# Autodesk Inventor assembly: Shipping goods QR subassembly
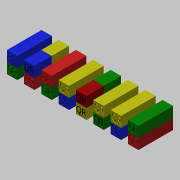
[picture p0: Inventor's stored thumbnail of the model, 180x180]
Saved by Autodesk Inventor 2015 (Build 190159000, 159)
## iProperties
Created: 2015-03-08
Part Number: Shipping goods QR subassembly
Document SubType Name: Assembly
Designer: Vukica
Author: Vukica
## Documents named in this file (9)
- D:\Dropbox\Dropbox\Service\IEEE\!Final Rules\2016Hardware_Court_v8-aug12\Shipping goods QR subassembly.iam
- D:\Dropbox\Dropbox\Service\IEEE\!Final Rules\2016Hardware_Court_v8-aug12\Container 2 2 5.ipt
- D:\Dropbox\Dropbox\Service\IEEE\!Final Rules\2016Hardware_Court_v8-aug12\Container 2 2 2 and half.ipt
- D:\Dropbox\Dropbox\Service\IEEE\!Final Rules\2016Hardware_Court_v8-aug12\Container 2 2 2 and half color 2.ipt
- D:\Dropbox\Dropbox\Service\IEEE\!Final Rules\2016Hardware_Court_v8-aug12\Container 2 2 2 and half color 4.ipt
- D:\Dropbox\Dropbox\Service\IEEE\!Final Rules\2016Hardware_Court_v8-aug12\Container 2 2 2 and half color 5.ipt
- D:\Dropbox\Dropbox\Service\IEEE\!Final Rules\2016Hardware_Court_v8-aug12\Container 2 2 5 QR color 5.ipt
- D:\Dropbox\Dropbox\Service\IEEE\!Final Rules\2016Hardware_Court_v8-aug12\Container 2 2 5 QR color 6.ipt
- D:\Dropbox\Dropbox\Service\IEEE\!Final Rules\2016Hardware_Court_v8-aug12\Container 2 2 5 QR color 2.ipt
## Components (20 placed, 8 different names)
1. Container 2 2 5:1 — Flush:1, Mate:1, Flush:2, Mate:4, Flush:6, Flush:8
2. Container 2 2 2 and half:1 — Flush:1, Mate:1, Flush:2, Mate:8, Mate:16, Mate:19
3. Container 2 2 2 and half color 4:1 — Mate:8
4. Container 2 2 5 QR color 5:1 — Mate:6, Flush:11, Flush:12, Mate:12, Flush:17, Flush:18
5. Container 2 2 5 QR color 2:1 — Mate:4, Flush:6, Flush:8, Mate:6, Flush:11, Flush:12, Mate:14
6. Container 2 2 2 and half:2 — Mate:13, Flush:19, Flush:20
7. Container 2 2 2 and half color 5:2 — Mate:12, Flush:17, Flush:18, Mate:13, Flush:19, Flush:20, Mate:15, Flush:21, Flush:27
8. Container 2 2 2 and half color 4:2 — Mate:18, Flush:23, Flush:24, Mate:19, Flush:25, Mate:22, Flush:26, Flush:50
9. Container 2 2 2 and half color 2:2 — Mate:18, Flush:23, Flush:24, Mate:20
10. Container 2 2 5 QR color 6:2 — Mate:16, Mate:17, Flush:22, Mate:20, Flush:25
11. Container 2 2 5 QR color 5:2 — Mate:14, Mate:15, Flush:21, Mate:17, Flush:22
12. Container 2 2 5 QR color 6:3 — Mate:22, Flush:26, Mate:30, Flush:40, Flush:41, Flush:42, Flush:44, Flush:48, Mate:33, Flush:50
13. Container 2 2 5:2 — Flush:27, Mate:28, Flush:36, Flush:37
14. Container 2 2 5 QR color 2:3 — Mate:28, Flush:36, Flush:37
15. Container 2 2 2 and half color 2:3 — Mate:29, Flush:38, Flush:39, Mate:30, Flush:40, Flush:41, Flush:43, Flush:45
16. Container 2 2 2 and half color 5:3 — Mate:29, Flush:38, Flush:39
17. Container 2 2 5:3 — Flush:43, Mate:31, Flush:47
18. Container 2 2 5 QR color 6:4 — Flush:42, Mate:31, Flush:47, Flush:48, Flush:49, Mate:33, Mate:34
19. Container 2 2 5 QR color 5:3 — Flush:45, Mate:32, Flush:46, Mate:34
20. Container 2 2 5 QR color 2:4 — Flush:44, Mate:32, Flush:46, Flush:49
## Relationships (53: Flush 32, Mate 21)
- Flush:1: Container 2 2 5:1 ↔ Container 2 2 2 and half:1
- Mate:1 (25.4 mm): Container 2 2 5:1 ↔ Container 2 2 2 and half:1
- Flush:2: Container 2 2 5:1 ↔ Container 2 2 2 and half:1
- Mate:4 (25.4 mm): Container 2 2 5:1 ↔ Container 2 2 5 QR color 2:1
- Flush:6: Container 2 2 5:1 ↔ Container 2 2 5 QR color 2:1
- Flush:8: Container 2 2 5:1 ↔ Container 2 2 5 QR color 2:1
- Mate:6 (25.4 mm): Container 2 2 5 QR color 5:1 ↔ Container 2 2 5 QR color 2:1
- Flush:11: Container 2 2 5 QR color 5:1 ↔ Container 2 2 5 QR color 2:1
- Flush:12: Container 2 2 5 QR color 5:1 ↔ Container 2 2 5 QR color 2:1
- Mate:8: Container 2 2 2 and half:1 ↔ Container 2 2 2 and half color 4:1
- Mate:12: Container 2 2 5 QR color 5:1 ↔ Container 2 2 2 and half color 5:2
- Flush:17: Container 2 2 5 QR color 5:1 ↔ Container 2 2 2 and half color 5:2
- Flush:18: Container 2 2 5 QR color 5:1 ↔ Container 2 2 2 and half color 5:2
- Mate:13: Container 2 2 2 and half:2 ↔ Container 2 2 2 and half color 5:2
- Flush:19: Container 2 2 2 and half:2 ↔ Container 2 2 2 and half color 5:2
- Flush:20: Container 2 2 2 and half:2 ↔ Container 2 2 2 and half color 5:2
- Mate:14: Container 2 2 5 QR color 2:1 ↔ Container 2 2 5 QR color 5:2
- Mate:15 (25.4 mm): Container 2 2 2 and half color 5:2 ↔ Container 2 2 5 QR color 5:2
- Flush:21: Container 2 2 2 and half color 5:2 ↔ Container 2 2 5 QR color 5:2
- Mate:16: Container 2 2 2 and half:1 ↔ Container 2 2 5 QR color 6:2
- Mate:17 (25.4 mm): Container 2 2 5 QR color 6:2 ↔ Container 2 2 5 QR color 5:2
- Flush:22: Container 2 2 5 QR color 6:2 ↔ Container 2 2 5 QR color 5:2
- Mate:18: Container 2 2 2 and half color 4:2 ↔ Container 2 2 2 and half color 2:2
- Flush:23: Container 2 2 2 and half color 4:2 ↔ Container 2 2 2 and half color 2:2
- Flush:24: Container 2 2 2 and half color 4:2 ↔ Container 2 2 2 and half color 2:2
- Mate:19: Container 2 2 2 and half:1 ↔ Container 2 2 2 and half color 4:2
- Mate:20 (25.4 mm): Container 2 2 2 and half color 2:2 ↔ Container 2 2 5 QR color 6:2
- Flush:25: Container 2 2 2 and half color 4:2 ↔ Container 2 2 5 QR color 6:2
- Mate:22 (25.4 mm): Container 2 2 2 and half color 4:2 ↔ Container 2 2 5 QR color 6:3
- Flush:26: Container 2 2 2 and half color 4:2 ↔ Container 2 2 5 QR color 6:3
- Flush:27: Container 2 2 2 and half color 5:2 ↔ Container 2 2 5:2
- Mate:28: Container 2 2 5:2 ↔ Container 2 2 5 QR color 2:3
- Flush:36: Container 2 2 5:2 ↔ Container 2 2 5 QR color 2:3
- Flush:37: Container 2 2 5:2 ↔ Container 2 2 5 QR color 2:3
- Mate:29: Container 2 2 2 and half color 2:3 ↔ Container 2 2 2 and half color 5:3
- Flush:38: Container 2 2 2 and half color 2:3 ↔ Container 2 2 2 and half color 5:3
- Flush:39: Container 2 2 2 and half color 2:3 ↔ Container 2 2 2 and half color 5:3
- Mate:30: Container 2 2 5 QR color 6:3 ↔ Container 2 2 2 and half color 2:3
- Flush:40: Container 2 2 5 QR color 6:3 ↔ Container 2 2 2 and half color 2:3
- Flush:41: Container 2 2 5 QR color 6:3 ↔ Container 2 2 2 and half color 2:3
- Flush:42: Container 2 2 5 QR color 6:3 ↔ Container 2 2 5 QR color 6:4
- Flush:43: Container 2 2 2 and half color 2:3 ↔ Container 2 2 5:3
- Flush:44: Container 2 2 5 QR color 6:3 ↔ Container 2 2 5 QR color 2:4
- Flush:45: Container 2 2 2 and half color 2:3 ↔ Container 2 2 5 QR color 5:3
- Mate:31: Container 2 2 5:3 ↔ Container 2 2 5 QR color 6:4
- Mate:32: Container 2 2 5 QR color 5:3 ↔ Container 2 2 5 QR color 2:4
- Flush:46: Container 2 2 5 QR color 5:3 ↔ Container 2 2 5 QR color 2:4
- Flush:47: Container 2 2 5:3 ↔ Container 2 2 5 QR color 6:4
- Flush:48: Container 2 2 5 QR color 6:3 ↔ Container 2 2 5 QR color 6:4
- Flush:49: Container 2 2 5 QR color 6:4 ↔ Container 2 2 5 QR color 2:4
- Mate:33 (25.4 mm): Container 2 2 5 QR color 6:3 ↔ Container 2 2 5 QR color 6:4
- Mate:34 (25.4 mm): Container 2 2 5 QR color 6:4 ↔ Container 2 2 5 QR color 5:3
- Flush:50: Container 2 2 2 and half color 4:2 ↔ Container 2 2 5 QR color 6:3
